# Autodesk Inventor assembly: AASTRC Top case cover
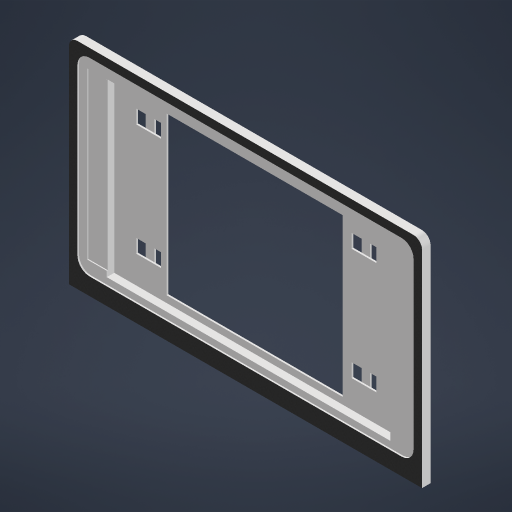
[picture p0: Inventor's stored thumbnail of the model, 512x512]
Saved by Autodesk Inventor 2024.2 (Build 282272000, 272)
## iProperties
Created: 2023-07-17
Part Number: AASTRC Top case cover
Document SubType Name: Assembly
Designer: wodyd
Author: wodyd
## Documents named in this file (4)
- C:\Users\6gioc\OneDrive\AAST\PART\AAST Remote Controler\AASTRC Top case cover.iam
- C:\Users\6gioc\OneDrive\AAST\PART\AAST Remote Controler\AASTRC Top case cover.ipt
- C:\Users\6gioc\OneDrive\AAST\PART\AAST Remote Controler\Raspberry Pi Display V1.1\Raspberry Pi Display V1.1.ipt
- C:\Users\6gioc\OneDrive\AAST\PART\AAST Remote Controler\display lock pin.ipt
## Components (4 placed, 3 different names)
1. AASTRC Top case cover:1 — 강체:1
2. Raspberry Pi Display V1.1:1 — 강체:1, 강체:2, 강체:3
3. display lock pin:1 — 강체:2
4. display lock pin:2 — 강체:3
## Relationships (3: WeldJoint 3)
- 강체:1 [WeldJoint]: AASTRC Top case cover:1 ↔ Raspberry Pi Display V1.1:1
- 강체:2 [WeldJoint]: Raspberry Pi Display V1.1:1 ↔ display lock pin:1
- 강체:3 [WeldJoint]: Raspberry Pi Display V1.1:1 ↔ display lock pin:2
